# Autodesk Inventor assembly: foot type 3
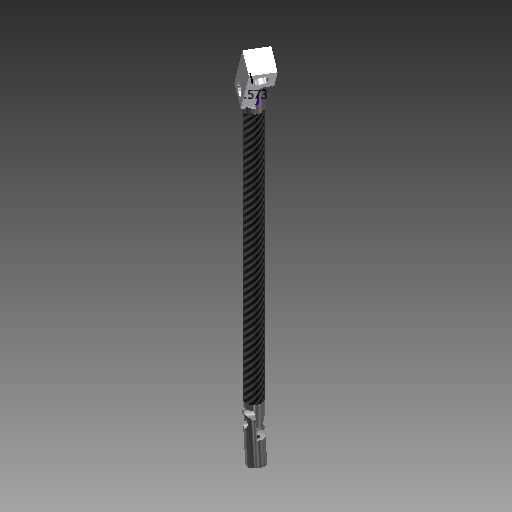
[picture p0: Inventor's stored thumbnail of the model, 512x512]
Saved by Autodesk Inventor 2018 (Build 220112000, 112)
## iProperties
Created: 2018-10-16
Part Number: foot type 3
Document SubType Name: Assembly
Designer: freyja
Author: freyja
## Documents named in this file (5)
- C:\Users\freyja\Documents\Cryostat\CAD\foot type 3.iam
- C:\Users\freyja\Documents\Cryostat\CAD\feet type 3 part 1.ipt
- C:\Users\freyja\Documents\Cryostat\CAD\feet type 3 part 2.ipt
- C:\Users\freyja\Documents\Cryostat\CAD\feet type 3 part 3.ipt
- C:\Users\freyja\Documents\Cryostat\CAD\mount.ipt
## Components (5 placed, 4 different names)
1. feet type 3 part 1:1 — Mate:2, Mate:4, Flush:1
2. feet type 3 part 2:1 — Mate:7, Mate:8, Mate:9, Mate:10
3. feet type 3 part 3:1 — Mate:5, Mate:6, Mate:7, Mate:8
4. feet type 3 part 2:2 — Mate:2, Mate:4, Mate:5, Mate:6
5. mount:1 — Mate:9, Mate:10, Flush:1
## Relationships (9: Mate 8, Flush 1)
- Mate:2: feet type 3 part 1:1 ↔ feet type 3 part 2:2
- Mate:4: feet type 3 part 1:1 ↔ feet type 3 part 2:2
- Mate:5: feet type 3 part 3:1 ↔ feet type 3 part 2:2
- Mate:6: feet type 3 part 3:1 ↔ feet type 3 part 2:2
- Mate:7: feet type 3 part 2:1 ↔ feet type 3 part 3:1
- Mate:8: feet type 3 part 2:1 ↔ feet type 3 part 3:1
- Mate:9: feet type 3 part 2:1 ↔ mount:1
- Mate:10: feet type 3 part 2:1 ↔ mount:1
- Flush:1: feet type 3 part 1:1 ↔ mount:1
